# Autodesk Inventor assembly: Joshuas Mistakes
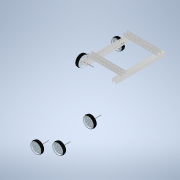
[picture p0: Inventor's stored thumbnail of the model, 180x180]
Saved by Autodesk Inventor 2020.1 (Build 241239000, 239)
## iProperties
Created: 2019-09-10
Part Number: Joshuas Mistakes
Document SubType Name: Assembly
Designer: alphaomega
Author: alphaomega
## Documents named in this file (9)
- B:\Documents\GitHub\AO_Robotics\CAD\Projects\Joshua Schmidt\Joshuas Mistakes.iam
- B:\Documents\GitHub\AO_Robotics\CAD\Parts Kits\FTC Tetrix KOP Organized (7-24-19)\Frame Hardware\Tetrix_39069.ipt
- B:\Documents\GitHub\AO_Robotics\CAD\Parts Kits\FTC Tetrix KOP Organized (7-24-19)\Frame Hardware\Tetrix_39068.ipt
- B:\Documents\GitHub\AO_Robotics\CAD\Parts Kits\FTC Tetrix KOP Organized (7-24-19)\Axle Hardware\Tetrix_39091.ipt
- B:\Documents\GitHub\AO_Robotics\CAD\Parts Kits\FTC Tetrix KOP Organized (7-24-19)\Axle Hardware\Tetrix_39172.iam
- B:\Documents\GitHub\AO_Robotics\CAD\Parts Kits\FTC Tetrix KOP Organized (7-24-19)\Axle Hardware\Tetrix_39100.ipt
- B:\Documents\GitHub\AO_Robotics\CAD\Parts Kits\FTC Tetrix KOP Organized (7-24-19)\Axle Hardware\Tetrix_39092.iam
- B:\Documents\GitHub\AO_Robotics\CAD\Parts Kits\FTC Tetrix KOP Organized (7-24-19)\Axle Hardware\Tetrix_39088.ipt
- B:\Documents\GitHub\AO_Robotics\CAD\Parts Kits\FTC Tetrix KOP Organized (7-24-19)\Wheel\Tetrix_39055.ipt
## Components (27 placed, 8 different names)
1. Tetrix_39069:1 — Rigid:2, Rotational:1, Flush:1
2. Tetrix_39068:1 — Rigid:2, Rigid:3
3. Tetrix_39069:2 — Rigid:3, Rigid:19, Rigid:20
4. Tetrix_39068:2 — Rotational:1, Flush:1
5. Tetrix_39091:1 — Rigid:19, Rotational:2
6. Tetrix_39091:2 — Rigid:20, Rotational:3
7. Tetrix_39172:1 [sub-assembly] — Rigid:5, Rigid:6
8. Tetrix_39100:1 — Rigid:6, Rotational:2
9. Tetrix_39092:1 [sub-assembly] — Rotational:3
10. Tetrix_39088:1 — Rigid:4
11. Tetrix_39055:1 — Rigid:4, Rigid:5
12. Tetrix_39172:2 [sub-assembly]
13. Tetrix_39100:2
14. Tetrix_39088:2
15. Tetrix_39055:2
16. Tetrix_39172:3 [sub-assembly]
17. Tetrix_39100:3
18. Tetrix_39088:3
19. Tetrix_39055:3
20. Tetrix_39172:4 [sub-assembly]
21. Tetrix_39100:4
22. Tetrix_39088:4
23. Tetrix_39055:4
24. Tetrix_39172:5 [sub-assembly]
25. Tetrix_39100:5
26. Tetrix_39088:5
27. Tetrix_39055:5
## Relationships (23: WeldJoint 19, RevoluteJoint 3, Flush 1)
- Rigid:2 [WeldJoint]: Tetrix_39069:1 ↔ Tetrix_39068:1
- Rotational:1 [RevoluteJoint]: Tetrix_39069:1 ↔ Tetrix_39068:2
- Flush:1: Tetrix_39069:1 ↔ Tetrix_39068:2
- Rigid:3 [WeldJoint]: Tetrix_39068:1 ↔ Tetrix_39069:2
- Rigid:4 [WeldJoint]: Tetrix_39088:1 ↔ Tetrix_39055:1
- Rigid:5 [WeldJoint]: Tetrix_39172:1 ↔ Tetrix_39055:1
- Rigid:6 [WeldJoint]: Tetrix_39172:1 ↔ Tetrix_39100:1
- [WeldJoint]: Tetrix_39088:2 ↔ Tetrix_39055:2
- [WeldJoint]: Tetrix_39172:2 ↔ Tetrix_39055:2
- [WeldJoint]: Tetrix_39172:2 ↔ Tetrix_39100:2
- [WeldJoint]: Tetrix_39088:3 ↔ Tetrix_39055:3
- [WeldJoint]: Tetrix_39172:3 ↔ Tetrix_39055:3
- [WeldJoint]: Tetrix_39172:3 ↔ Tetrix_39100:3
- [WeldJoint]: Tetrix_39088:4 ↔ Tetrix_39055:4
- [WeldJoint]: Tetrix_39172:4 ↔ Tetrix_39055:4
- [WeldJoint]: Tetrix_39172:4 ↔ Tetrix_39100:4
- [WeldJoint]: Tetrix_39088:5 ↔ Tetrix_39055:5
- [WeldJoint]: Tetrix_39172:5 ↔ Tetrix_39055:5
- [WeldJoint]: Tetrix_39172:5 ↔ Tetrix_39100:5
- Rigid:19 [WeldJoint]: Tetrix_39069:2 ↔ Tetrix_39091:1
- Rigid:20 [WeldJoint]: Tetrix_39069:2 ↔ Tetrix_39091:2
- Rotational:2 [RevoluteJoint]: Tetrix_39091:1 ↔ Tetrix_39100:1
- Rotational:3 [RevoluteJoint]: Tetrix_39091:2 ↔ Tetrix_39092:1
## Named parameters: d21_d18 = 0 mm, d22_d19 = 0 mm, d23_d20 = 0 mm, d24_d18 = 0 mm, d25_d19 = 0 mm, d26_d20 = 0 mm, d27_d18 = 0 mm, d28_d19 = 0 mm, d29_d20 = 0 mm, d30_d18 = 0 mm, d31_d19 = 0 mm, d32_d20 = 0 mm
